# Autodesk Inventor assembly: CNC_X6
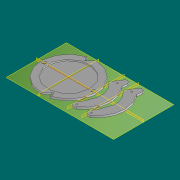
[picture p0: Inventor's stored thumbnail of the model, 180x180]
Saved by Autodesk Inventor 2022 (Build 260153000, 153)
## iProperties
Created: 2023-06-04
Part Number: CNC_X6
Document SubType Name: Assembly
Designer: gisen
Author: gisen
## Documents named in this file (3)
- C:\Users\gisen\Documents\CAD\inventor\git\cook\canere\CNC_X6.iam
- C:\Users\gisen\Documents\CAD\inventor\git\cook\canere\canere_01.ipt
- C:\Users\gisen\Documents\CAD\inventor\git\cook\canere\canere_02_t3_01.ipt
## Components (3 placed, 2 different names)
1. canere_01:1
2. canere_02_t3_01:1 — メイト:1, メイト:3, フラッシュ:1, メイト:4
3. canere_02_t3_01:2 — メイト:2, フラッシュ:1, メイト:5
## Relationships (6: Mate 5, Flush 1)
- メイト:1 [Mate]: canere_02_t3_01:1
- メイト:2 [Mate]: canere_02_t3_01:2
- メイト:3 [Mate] (41 mm): canere_02_t3_01:1
- フラッシュ:1 [Flush] (23 mm): canere_02_t3_01:1 ↔ canere_02_t3_01:2
- メイト:4 [Mate]: canere_02_t3_01:1
- メイト:5 [Mate]: canere_02_t3_01:2
